# Autodesk Inventor assembly: head
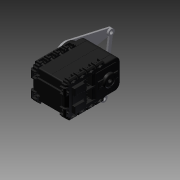
[picture p0: Inventor's stored thumbnail of the model, 180x180]
Saved by Autodesk Inventor 2013 SP2 (Build 170200200, 200)
## iProperties
Created: 2014-11-25
Part Number: head
Document SubType Name: Assembly
Designer: Master
Author: Master
## Documents named in this file (4)
- C:\Users\Master\Documents\GitHub\DIY-HR-OS1\CAD Files\head.iam
- C:\Users\Master\Documents\GitHub\DIY-HR-OS1\CAD Files\AX12\AX12.iam
- C:\Users\Master\Documents\GitHub\DIY-HR-OS1\CAD Files\headtilt-teardrop.ipt
- C:\Users\Master\Documents\GitHub\DIY-HR-OS1\CAD Files\headtilt-long.ipt
## Components (3 placed, 3 different names)
1. AX12:1 [sub-assembly] — Mate:1, Mate:2, Mate:3, Mate:4
2. headtilt-teardrop:1 — Mate:3, Mate:4, Mate:5, Mate:6
3. headtilt-long:1 — Mate:5, Mate:6
## Relationships (6: Mate 6)
- Mate:1: AX12:1
- Mate:2: AX12:1
- Mate:3: AX12:1 ↔ headtilt-teardrop:1
- Mate:4: AX12:1 ↔ headtilt-teardrop:1
- Mate:5: headtilt-teardrop:1 ↔ headtilt-long:1
- Mate:6: headtilt-teardrop:1 ↔ headtilt-long:1
